# Autodesk Inventor assembly: Enclave
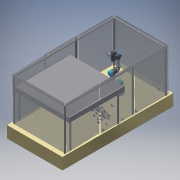
[picture p0: Inventor's stored thumbnail of the model, 180x180]
Saved by Autodesk Inventor 2017 (Build 210142000, 142)
## iProperties
Created: 2017-06-26
Part Number: Enclave
Document SubType Name: Assembly
Designer: sensor
Author: sensor
## Documents named in this file (11)
- C:\Users\sensor\Documents\JB's Work\Enclave.iam
- C:\Users\sensor\Documents\JB's Work\20 2020 2andhalffoot.ipt
- C:\Users\sensor\Documents\JB's Work\20 2020.ipt
- C:\Users\sensor\Documents\JB's Work\20 2020 3ft.ipt
- C:\Users\sensor\Documents\JB's Work\20 2020 1andahalfft.ipt
- C:\Users\sensor\Documents\JB's Work\Table.ipt
- C:\Users\sensor\Documents\JB's Work\Sketchy Robot Site\62973032-9-ur3\ur3.iam
- C:\Users\sensor\Documents\JB's Work\XCarve.ipt
- C:\Users\sensor\Documents\JB's Work\PlexiglassWall2ft.ipt
- C:\Users\sensor\Documents\JB's Work\PlexiglassWall3ft.ipt
- C:\Users\sensor\Documents\JB's Work\Brackket.ipt
## Components (97 placed, 10 different names)
1. 20 2020 2andhalffoot:1
2. 20 2020 2andhalffoot:2 — Mate:9
3. 20 2020:1
4. 20 2020:2
5. 20 2020 2andhalffoot:3
6. 20 2020 2andhalffoot:4
7. 20 2020 3ft:1
8. 20 2020 3ft:2
9. 20 2020 1andahalfft:1
10. 20 2020 1andahalfft:2
11. 20 2020 1andahalfft:3 — Mate:3
12. 20 2020 1andahalfft:4
13. Table:1 — Mate:1, Mate:2, Mate:3, Mate:4, Mate:5, Mate:6, Mate:7, Mate:8, Mate:9
14. ur3:1 [sub-assembly]
15. 20 2020 3ft:3
16. 20 2020 3ft:4
17. XCarve:1
18. 20 2020 2andhalffoot:5 — Mate:5
19. 20 2020 2andhalffoot:6
20. PlexiglassWall2ft:1
21. PlexiglassWall2ft:2
22. PlexiglassWall2ft:3
23. PlexiglassWall2ft:4
24. PlexiglassWall2ft:5
25. PlexiglassWall2ft:6
26. PlexiglassWall3ft:1
27. PlexiglassWall3ft:2
28. Brackket:1
29. Brackket:2
30. Brackket:3 — Insert:1
31. Brackket:4 — Insert:1
32. Brackket:5
33. Brackket:6 — Mate:8
34. Brackket:7
35. Brackket:8
36. Brackket:9
37. Brackket:10
38. Brackket:11
39. Brackket:12
40. Brackket:13
41. Brackket:14
42. Brackket:15
43. Brackket:16
44. Brackket:17
45. Brackket:18
46. Brackket:19
47. Brackket:20
48. Brackket:21
49. Brackket:22
50. Brackket:23
51. Brackket:24 — Mate:1
52. Brackket:25
53. Brackket:26
54. Brackket:27
55. Brackket:28
56. Brackket:29
57. Brackket:30
58. Brackket:31
59. Brackket:32
60. Brackket:33
61. Brackket:34
62. Brackket:35
63. Brackket:36
64. Brackket:37
65. Brackket:38
66. Brackket:39
67. Brackket:40
68. Brackket:41
69. Brackket:42
70. Brackket:43
71. Brackket:44
72. Brackket:45
73. Brackket:46
74. Brackket:47
75. Brackket:48
76. Brackket:49 — Mate:2
77. Brackket:50 — Mate:7
78. Brackket:51
79. Brackket:52
80. Brackket:53 — Mate:4
81. Brackket:54
82. Brackket:55
83. Brackket:56
84. Brackket:57
85. Brackket:58
86. Brackket:59
87. Brackket:60
88. Brackket:61 — Mate:6
89. Brackket:62
90. Brackket:63
91. Brackket:64
92. Brackket:65
93. Brackket:66
94. Brackket:67
95. Brackket:68
96. Brackket:69
97. Brackket:70
## Relationships (10: Mate 9, Insert 1)
- Insert:1: Brackket:3 ↔ Brackket:4
- Mate:1: Table:1 ↔ Brackket:24
- Mate:2: Table:1 ↔ Brackket:49
- Mate:3: 20 2020 1andahalfft:3 ↔ Table:1
- Mate:4: Table:1 ↔ Brackket:53
- Mate:5: Table:1 ↔ 20 2020 2andhalffoot:5
- Mate:6: Table:1 ↔ Brackket:61
- Mate:7: Table:1 ↔ Brackket:50
- Mate:8: Table:1 ↔ Brackket:6
- Mate:9: 20 2020 2andhalffoot:2 ↔ Table:1
